# Autodesk Inventor assembly: SM_ZA01
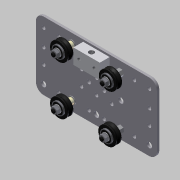
[picture p0: Inventor's stored thumbnail of the model, 180x180]
Saved by Autodesk Inventor 2012 SP1 (Build 160190100, 190)
## iProperties
Created: 2012-05-01
Part Number: SM_ZA01
Document SubType Name: Assembly
Designer: ERF
Stock Number: SM_ZA01
Author: ERF
Title: Z Axis Mount Plate Assembly
## Documents named in this file (10)
- C:\Users\eford\Documents\Projects\Shapoko_v1i\Workspaces\Workspace\Projects\USER FOLDER\Edward\Shapeoko_v1i\Assemblies\SM-ZA01.iam
- C:\Users\eford\Documents\Projects\Shapoko_v1i\Workspaces\Workspace\Projects\USER FOLDER\Edward\Shapeoko_v1i\Parts\MSK01-01.ipt
- C:\Users\eford\Documents\Projects\Shapoko_v1i\Workspaces\Workspace\Projects\USER FOLDER\Edward\Shapeoko_v1i\Parts\SM-M08.ipt
- C:\Users\eford\Documents\Projects\Shapoko_v1i\Workspaces\Workspace\Projects\USER FOLDER\Edward\Shapeoko_v1i\Parts\MSK01-04.ipt
- C:\Users\eford\Documents\Projects\Shapoko_v1i\Workspaces\Workspace\Projects\USER FOLDER\Edward\Shapeoko_v1i\Parts\SM-H04.ipt
- C:\Users\eford\Documents\Projects\Shapoko_v1i\Workspaces\Workspace\Projects\USER FOLDER\Edward\Shapeoko_v1i\Parts\SM-H01.ipt
- C:\Users\eford\Documents\Projects\Shapoko_v1i\Workspaces\Workspace\Projects\USER FOLDER\Edward\Shapeoko_v1i\Parts\SM-H03.ipt
- C:\Users\eford\Documents\Projects\Shapoko_v1i\Workspaces\Workspace\Projects\USER FOLDER\Edward\Shapeoko_v1i\Parts\SM-H08.ipt
- C:\Users\eford\Documents\Projects\Shapoko_v1i\Workspaces\Workspace\Projects\USER FOLDER\Edward\Shapeoko_v1i\Parts\SM-H07.ipt
- C:\Users\eford\Documents\Projects\Shapoko_v1i\Workspaces\Workspace\Projects\USER FOLDER\Edward\Shapeoko_v1i\Assemblies\MSK01-05A.iam
## Components (36 placed, 9 different names)
1. MSK01-01:1 — Insert:4, Insert:5, Insert:9, Insert:10, Mate:2, Mate:4, Insert:12, Insert:13, Insert:33, Insert:34, Insert:35, Insert:36
2. MSK01-04:1 — Insert:9, Mate:3, Insert:14
3. MSK01-04:2 — Insert:10, Mate:1, Insert:11
4. SM-H04:1 — Insert:29
5. SM-H04:2 — Insert:30
6. SM-H01:1 — Insert:15, Insert:17
7. SM-H01:2 — Insert:16, Insert:18
8. SM-H03:1 — Insert:7, Mate:4
9. SM-H08:1 — Insert:7, Mate:3
10. SM-H03:2 — Insert:1, Mate:2
11. SM-H08:2 — Insert:1, Mate:1
12. SM-H03:3 — Insert:2, Insert:5
13. SM-H08:3 — Insert:2
14. SM-H03:4 — Insert:3, Insert:4
15. SM-H08:4 — Insert:3
16. SM-H03:5 — Insert:14, Insert:20
17. SM-H03:6 — Insert:13, Insert:16
18. SM-H03:7 — Insert:12, Insert:15
19. SM-H03:8 — Insert:11, Insert:19
20. SM-H03:9 — Insert:18, Insert:39
21. SM-H03:10 — Insert:17, Insert:38
22. SM-H03:11 — Insert:19, Insert:37
23. SM-H03:12 — Insert:20, Insert:40
24. SM-H03:13 — Insert:30, Insert:44
25. SM-H03:14 — Insert:32, Insert:41
26. SM-H03:15 — Insert:31, Insert:42
27. SM-H03:16 — Insert:29, Insert:43
28. SM-H04:5 — Insert:31
29. SM-H04:6 — Insert:32
30. SM-M08:2 — Insert:33, Insert:34
31. SM-H07:3 — Insert:36
32. SM-H07:4 — Insert:35
33. MSK01-05A:9 [sub-assembly] — Insert:37, Insert:43
34. MSK01-05A:10 [sub-assembly] — Insert:38, Insert:44
35. MSK01-05A:11 [sub-assembly] — Insert:39, Insert:41
36. MSK01-05A:12 [sub-assembly] — Insert:40, Insert:42
## Relationships (38: Insert 34, Mate 4)
- Insert:1: SM-H03:2 ↔ SM-H08:2
- Insert:2: SM-H03:3 ↔ SM-H08:3
- Insert:3: SM-H03:4 ↔ SM-H08:4
- Insert:4: MSK01-01:1 ↔ SM-H03:4
- Insert:5: MSK01-01:1 ↔ SM-H03:3
- Insert:7: SM-H03:1 ↔ SM-H08:1
- Insert:9: MSK01-01:1 ↔ MSK01-04:1
- Insert:10: MSK01-01:1 ↔ MSK01-04:2
- Mate:1: MSK01-04:2 ↔ SM-H08:2
- Mate:2: MSK01-01:1 ↔ SM-H03:2
- Mate:3: MSK01-04:1 ↔ SM-H08:1
- Mate:4: MSK01-01:1 ↔ SM-H03:1
- Insert:11: MSK01-04:2 ↔ SM-H03:8
- Insert:12: MSK01-01:1 ↔ SM-H03:7
- Insert:13: MSK01-01:1 ↔ SM-H03:6
- Insert:14: MSK01-04:1 ↔ SM-H03:5
- Insert:15: SM-H01:1 ↔ SM-H03:7
- Insert:16: SM-H01:2 ↔ SM-H03:6
- Insert:17: SM-H01:1 ↔ SM-H03:10
- Insert:18: SM-H01:2 ↔ SM-H03:9
- Insert:19: SM-H03:8 ↔ SM-H03:11
- Insert:20: SM-H03:5 ↔ SM-H03:12
- Insert:29: SM-H04:1 ↔ SM-H03:16
- Insert:30: SM-H04:2 ↔ SM-H03:13
- Insert:31: SM-H03:15 ↔ SM-H04:5
- Insert:32: SM-H03:14 ↔ SM-H04:6
- Insert:33: MSK01-01:1 ↔ SM-M08:2
- Insert:34: MSK01-01:1 ↔ SM-M08:2
- Insert:35: MSK01-01:1 ↔ SM-H07:4
- Insert:36: MSK01-01:1 ↔ SM-H07:3
- Insert:37: SM-H03:11 ↔ MSK01-05A:9
- Insert:38: SM-H03:10 ↔ MSK01-05A:10
- Insert:39: SM-H03:9 ↔ MSK01-05A:11
- Insert:40: SM-H03:12 ↔ MSK01-05A:12
- Insert:41: SM-H03:14 ↔ MSK01-05A:11
- Insert:42: SM-H03:15 ↔ MSK01-05A:12
- Insert:43: SM-H03:16 ↔ MSK01-05A:9
- Insert:44: SM-H03:13 ↔ MSK01-05A:10
